# Autodesk Inventor assembly: Placed corner cabinet concept
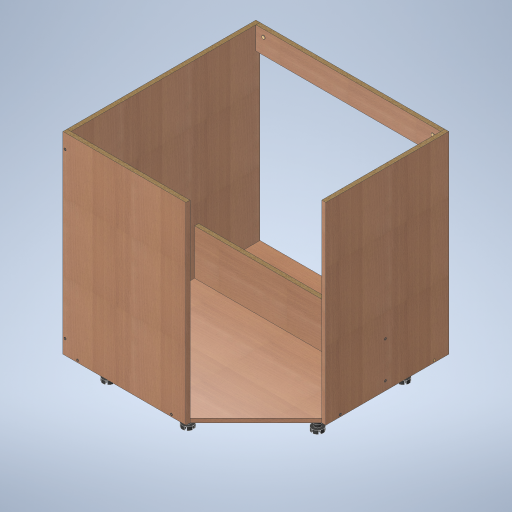
[picture p0: Inventor's stored thumbnail of the model, 512x512]
Saved by Autodesk Inventor 2024 (Build 280153000, 153)
## iProperties
RuleStatus: InUse
Created: 2017-01-19
Part Number: Placed corner cabinet concept
Document SubType Name: Assembly
Designer: SvetlanaB
Author: SvetlanaB
## Documents named in this file (16)
- C:\W4INV 2024 Design\iBOX LIBRARY\Kitchen\Standing Cabinets\Corner cabinet\corner cabinet.iam
- C:\W4INV 2024 Design\iBOX LIBRARY\Kitchen\Standing Cabinets\Corner cabinet\Right panel.ipt
- C:\W4INV 2024 Design\iBOX LIBRARY\Kitchen\Standing Cabinets\Corner cabinet\Left panel.ipt
- C:\W4INV 2024 Design\iBOX LIBRARY\Kitchen\Standing Cabinets\Corner cabinet\Skeleton Panel3.ipt
- C:\W4INV 2024 Design\iBOX LIBRARY\Kitchen\Standing Cabinets\Corner cabinet\Skeleton Panel4.ipt
- C:\W4INV 2024 Design\iBOX LIBRARY\Kitchen\Standing Cabinets\Corner cabinet\Back panel.ipt
- C:\W4INV 2024 Design\iBOX LIBRARY\Kitchen\Standing Cabinets\Corner cabinet\Middle panel_1.ipt
- C:\W4INV 2024 Design\_LIBRARY\Fixed joints\Confirmat\CONFIRMAT\Confirmat L50 NB T18 PB T 18.ipt
- C:\W4INV 2024 Design\_LIBRARY\Supports and legs\Legs\ADJUSTABLE LEG\Adjustable leg  BT18.ipt
- C:\W4INV 2024 Design\iBOX LIBRARY\Kitchen\Standing Cabinets\Corner cabinet\cabinet concept.ipt
- C:\W4INV 2024 Design\_LIBRARY\Fixed joints\Minifix joint\MINIFIX D15 v2\Minifix D15 & Dowel L34 & Cap D15 PB T18 LH.ipt
- C:\W4INV 2024 Design\_LIBRARY\Fixed joints\Minifix joint\MINIFIX D15 v2\Minifix D15 & Dowel L34 & Cap D15 PB T18 RH.ipt
- C:\W4INV 2024 Design\_LIBRARY\Fixed joints\Confirmat\CONFIRMAT\Confirmat L50 & Cap D10 NB T18 PB T 18.ipt
- C:\W4INV 2023 Design\LIBRARY\Fixed joints\Confirmat\CONFIRMAT.ipt
- C:\W4INV 2023 Design\LIBRARY\Fixed joints\Minifix joint\MINIFIX D15 v2.ipt
- C:\W4INV 2023 Design\LIBRARY\Supports and legs\Legs\ADJUSTABLE LEG.ipt
## Components (26 placed, 12 different names)
1. @Skeleton
2. Right panel:1 — Flush:4, Flush:8, Flush:10, Front (Angle) Plane:1, Front (Angle) Plane:2, Nestled Board Plane:1, Nestled Board Plane:2, Nestled Board Plane:10, Nestled Board Plane:13, Nestled Board Plane:7
3. Front panel:1 — Flush:1, Flush:7, Flush:9, Nestled Board Plane:3, Nestled Board Plane:4, Nestled Board Plane:11, Nestled Board Plane:12
4. Bottom panel:1 — Flush:5, Bottom board Plane:1, Bottom board Plane:2, Bottom board Plane:5, Bottom board Plane:3, Bottom board Plane:4, Pillar Board Side Plane:1, Pillar Board Side Plane:2, Pillar Board Side Plane:3, Pillar Board Side Plane:4, Pillar Board Side Plane:5, Pillar Board Side Plane:6
5. Left Panel:1 — Flush:2, Flush:3, Flush:21, Flush:30, Nestled Board Plane:5, Nestled Board Plane:6, Nestled Board Plane:9, Flush:37, Flush:38, Pillar Board Side Plane:11, Pillar Board Side Plane:12, Nestled Board Plane:14, Nestled Board Plane:8
6. Back link:1 — Flush:11, Flush:45, Pillar Board Side Plane :1, Pillar Board Side Plane :2
7. Adjustable leg  BT18:1 — Bottom board Plane:1, Axis Plane:1, Axis2 Plane:1
8. Adjustable leg  BT18:2 — Bottom board Plane:2, Axis Plane:2, Axis2 Plane:2
9. Adjustable leg  BT18:5 — Bottom board Plane:5, Axis Plane:5, Axis2 Plane:5
10. Middle shore:1 — Flush:25, Pillar Board Side Plane:9, Pillar Board Side Plane:10, Flush:42, Pillar Board Side Plane:13, Pillar Board Side Plane:14
11. Adjustable leg  BT18:6 — Axis Plane:3, Bottom board Plane:3, Axis2 Plane:3, Front (Angle) Plane:1
12. Adjustable leg  BT18:7 — Axis Plane:4, Bottom board Plane:4, Axis2 Plane:4, Front (Angle) Plane:2
13. Confirmat L50 & Cap D10 NB T18 PB T 18:1 — Axis Plane:6, Nestled Board Plane:1, Pillar Board Side Plane:1
14. Confirmat L50 NB T18 PB T 18:2 — Axis Plane:7, Nestled Board Plane:2, Pillar Board Side Plane:2
15. Confirmat L50 NB T18 PB T 18:3 — Axis Plane:8, Pillar Board Side Plane:3, Nestled Board Plane:3
16. Confirmat L50 NB T18 PB T 18:4 — Axis Plane:9, Pillar Board Side Plane:4, Nestled Board Plane:4
17. Confirmat L50 NB T18 PB T 18:5 — Axis Plane:10, Nestled Board Plane:5, Pillar Board Side Plane:5
18. Confirmat L50 NB T18 PB T 18:6 — Axis Plane:11, Nestled Board Plane:6, Pillar Board Side Plane:6
19. Confirmat L50 NB T18 PB T 18:9 — Nestled Board Plane:9, Pillar Board Side Plane:9, Axis Plane:14
20. Confirmat L50 NB T18 PB T 18:10 — Nestled Board Plane:10, Pillar Board Side Plane:10, Axis Plane:15
21. Confirmat L50 NB T18 PB T 18:11 — Axis Plane:16, Nestled Board Plane:11, Pillar Board Side Plane:11
22. Confirmat L50 NB T18 PB T 18:12 — Axis Plane:17, Nestled Board Plane:12, Pillar Board Side Plane:12
23. Confirmat L50 NB T18 PB T 18:13 — Nestled Board Plane:13, Pillar Board Side Plane:13, Axis Plane:18
24. Confirmat L50 NB T18 PB T 18:14 — Nestled Board Plane:14, Pillar Board Side Plane:14, Axis Plane:19
25. Minifix D15 & Dowel L34 & Cap D15 PB T18 LH:1 — Nestled Board Plane:7, Pillar Board Side Plane :1, Axis Plane:12
26. Minifix D15 & Dowel L34 & Cap D15 PB T18 RH:2 — Nestled Board Plane:8, Pillar Board Side Plane :2, Axis Plane:13
## Relationships (76: Mate 43, Flush 31, Angle 2)
- Flush:1 (-100 mm): Front panel:1
- Flush:2 (-100 mm): Left Panel:1
- Flush:3 (-450 mm): Left Panel:1
- Flush:4 (-100 mm): Right panel:1
- Flush:5 (-100 mm): Bottom panel:1
- Bottom board Plane:1 [Mate]: Bottom panel:1 ↔ Adjustable leg  BT18:1
- Axis Plane:1 [Mate]: Adjustable leg  BT18:1
- Axis2 Plane:1 [Mate]: Adjustable leg  BT18:1
- Bottom board Plane:2 [Mate]: Bottom panel:1 ↔ Adjustable leg  BT18:2
- Axis Plane:2 [Mate]: Adjustable leg  BT18:2
- Axis2 Plane:2 [Mate]: Adjustable leg  BT18:2
- Bottom board Plane:5 [Mate]: Bottom panel:1 ↔ Adjustable leg  BT18:5
- Axis Plane:5 [Mate]: Adjustable leg  BT18:5
- Axis2 Plane:5 [Mate]: Adjustable leg  BT18:5
- Flush:7 (-64 mm): Front panel:1
- Flush:8 (-64 mm): Right panel:1
- Flush:9 (-64 mm): Front panel:1
- Flush:10 (-64 mm): Right panel:1
- Flush:11 (-20 mm): Back link:1
- Flush:21 (-64 mm): Left Panel:1
- Flush:25 (-20 mm): Middle shore:1
- Axis Plane:3 [Mate]: Adjustable leg  BT18:6
- Bottom board Plane:3 [Mate]: Bottom panel:1 ↔ Adjustable leg  BT18:6
- Axis2 Plane:3 [Mate]: Adjustable leg  BT18:6
- Front (Angle) Plane:1 [Angle] (0 deg): Right panel:1 ↔ Adjustable leg  BT18:6
- Axis Plane:4 [Mate]: Adjustable leg  BT18:7
- Bottom board Plane:4 [Mate]: Bottom panel:1 ↔ Adjustable leg  BT18:7
- Axis2 Plane:4 [Mate]: Adjustable leg  BT18:7
- Front (Angle) Plane:2 [Angle] (0 deg): Right panel:1 ↔ Adjustable leg  BT18:7
- Axis Plane:6 [Mate]: Confirmat L50 & Cap D10 NB T18 PB T 18:1
- Nestled Board Plane:1 [Flush]: Right panel:1 ↔ Confirmat L50 & Cap D10 NB T18 PB T 18:1
- Pillar Board Side Plane:1 [Mate] (-9 mm): Bottom panel:1 ↔ Confirmat L50 & Cap D10 NB T18 PB T 18:1
- Axis Plane:7 [Mate]: Confirmat L50 NB T18 PB T 18:2
- Nestled Board Plane:2 [Flush]: Right panel:1 ↔ Confirmat L50 NB T18 PB T 18:2
- Pillar Board Side Plane:2 [Mate] (-9 mm): Bottom panel:1 ↔ Confirmat L50 NB T18 PB T 18:2
- Axis Plane:8 [Mate]: Confirmat L50 NB T18 PB T 18:3
- Pillar Board Side Plane:3 [Mate] (-9 mm): Bottom panel:1 ↔ Confirmat L50 NB T18 PB T 18:3
- Nestled Board Plane:3 [Flush]: Front panel:1 ↔ Confirmat L50 NB T18 PB T 18:3
- Axis Plane:9 [Mate]: Confirmat L50 NB T18 PB T 18:4
- Pillar Board Side Plane:4 [Mate] (-9 mm): Bottom panel:1 ↔ Confirmat L50 NB T18 PB T 18:4
- Nestled Board Plane:4 [Flush]: Front panel:1 ↔ Confirmat L50 NB T18 PB T 18:4
- Flush:30 (-64 mm): Left Panel:1
- Axis Plane:10 [Mate]: Confirmat L50 NB T18 PB T 18:5
- Nestled Board Plane:5 [Flush]: Left Panel:1 ↔ Confirmat L50 NB T18 PB T 18:5
- Pillar Board Side Plane:5 [Mate] (-9 mm): Bottom panel:1 ↔ Confirmat L50 NB T18 PB T 18:5
- Axis Plane:11 [Mate]: Confirmat L50 NB T18 PB T 18:6
- Nestled Board Plane:6 [Flush]: Left Panel:1 ↔ Confirmat L50 NB T18 PB T 18:6
- Pillar Board Side Plane:6 [Mate] (-9 mm): Bottom panel:1 ↔ Confirmat L50 NB T18 PB T 18:6
- Nestled Board Plane:9 [Flush]: Left Panel:1 ↔ Confirmat L50 NB T18 PB T 18:9
- Pillar Board Side Plane:9 [Mate] (-9 mm): Middle shore:1 ↔ Confirmat L50 NB T18 PB T 18:9
- Axis Plane:14 [Mate]: Confirmat L50 NB T18 PB T 18:9
- Nestled Board Plane:10 [Flush]: Right panel:1 ↔ Confirmat L50 NB T18 PB T 18:10
- Pillar Board Side Plane:10 [Mate] (-9 mm): Middle shore:1 ↔ Confirmat L50 NB T18 PB T 18:10
- Axis Plane:15 [Mate]: Confirmat L50 NB T18 PB T 18:10
- Flush:37 (-64 mm): Left Panel:1
- Flush:38 (-64 mm): Left Panel:1
- Axis Plane:16 [Mate]: Confirmat L50 NB T18 PB T 18:11
- Nestled Board Plane:11 [Flush]: Front panel:1 ↔ Confirmat L50 NB T18 PB T 18:11
- Pillar Board Side Plane:11 [Mate] (-9 mm): Left Panel:1 ↔ Confirmat L50 NB T18 PB T 18:11
- Axis Plane:17 [Mate]: Confirmat L50 NB T18 PB T 18:12
- Nestled Board Plane:12 [Flush]: Front panel:1 ↔ Confirmat L50 NB T18 PB T 18:12
- Pillar Board Side Plane:12 [Mate] (-9 mm): Left Panel:1 ↔ Confirmat L50 NB T18 PB T 18:12
- Flush:42 (-180 mm): Middle shore:1
- Nestled Board Plane:13 [Flush]: Right panel:1 ↔ Confirmat L50 NB T18 PB T 18:13
- Pillar Board Side Plane:13 [Mate] (-9 mm): Middle shore:1 ↔ Confirmat L50 NB T18 PB T 18:13
- Axis Plane:18 [Mate]: Confirmat L50 NB T18 PB T 18:13
- Nestled Board Plane:14 [Flush]: Left Panel:1 ↔ Confirmat L50 NB T18 PB T 18:14
- Pillar Board Side Plane:14 [Mate] (-9 mm): Middle shore:1 ↔ Confirmat L50 NB T18 PB T 18:14
- Axis Plane:19 [Mate]: Confirmat L50 NB T18 PB T 18:14
- Flush:45 (-30 mm): Back link:1
- Nestled Board Plane:7 [Mate]: Right panel:1 ↔ Minifix D15 & Dowel L34 & Cap D15 PB T18 LH:1
- Pillar Board Side Plane :1 [Flush] (18 mm): Back link:1 ↔ Minifix D15 & Dowel L34 & Cap D15 PB T18 LH:1
- Axis Plane:12 [Mate]: Minifix D15 & Dowel L34 & Cap D15 PB T18 LH:1
- Nestled Board Plane:8 [Mate]: Left Panel:1 ↔ Minifix D15 & Dowel L34 & Cap D15 PB T18 RH:2
- Pillar Board Side Plane :2 [Flush] (18 mm): Back link:1 ↔ Minifix D15 & Dowel L34 & Cap D15 PB T18 RH:2
- Axis Plane:13 [Mate]: Minifix D15 & Dowel L34 & Cap D15 PB T18 RH:2
## Named parameters: Panel_thickness = 18 mm, Left_Attachment_Width = 560 mm, Right_Attachment_Width = 560 mm, Door_Space = 384.66609 mm, LeftAttachmentWidth = 560 mm, SpaceForDoor = 384.66609 mm
